# Autodesk Inventor assembly: Steam Engine Assembly
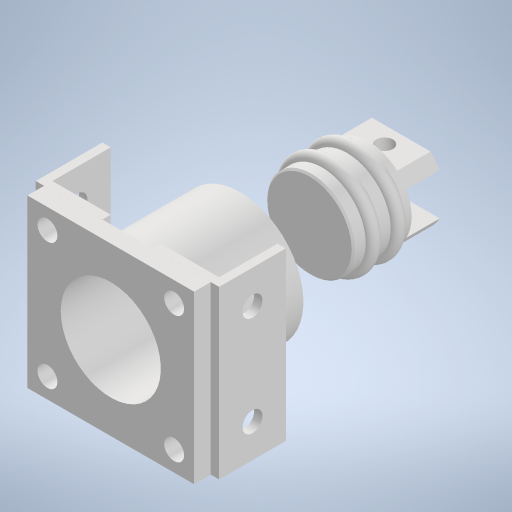
[picture p0: Inventor's stored thumbnail of the model, 512x512]
Saved by Autodesk Inventor 2023 (Build 270158000, 158)
## iProperties
Created: 2022-10-27
Part Number: Steam Engine Assembly
Document SubType Name: Assembly
Designer: tommy
Author: tommy
## Documents named in this file (5)
- C:\Users\tommy\Documents\Repositories\Steam Engine\Steam Engine Assembly.iam
- C:\Users\tommy\Documents\Repositories\Steam Engine\Cylinders.ipt
- C:\Users\tommy\Documents\Repositories\Steam Engine\Frame Bracket.ipt
- C:\Users\tommy\Documents\Repositories\Steam Engine\Piston.ipt
- C:\Users\tommy\Documents\Repositories\Steam Engine\Piston O Ring.ipt
## Components (6 placed, 4 different names)
1. Cylinders:1 — Mate:1, Mate:2, Mate:3, Mate:4, Mate:5, Mate:6, Mate:9
2. Frame Bracket:1 — Mate:1, Mate:3, Mate:4
3. Frame Bracket:2 — Mate:2, Mate:5, Mate:6
4. Piston:1 — Tangent:1, Tangent:2, Mate:7, Mate:8, Mate:9
5. Piston O Ring:1 — Tangent:2, Mate:8
6. Piston O Ring:2 — Tangent:1, Mate:7
## Relationships (11: Mate 9, Tangent 2)
- Mate:1: Cylinders:1 ↔ Frame Bracket:1
- Mate:2: Cylinders:1 ↔ Frame Bracket:2
- Mate:3: Cylinders:1 ↔ Frame Bracket:1
- Mate:4: Cylinders:1 ↔ Frame Bracket:1
- Mate:5: Cylinders:1 ↔ Frame Bracket:2
- Mate:6: Cylinders:1 ↔ Frame Bracket:2
- Tangent:1: Piston:1 ↔ Piston O Ring:2
- Tangent:2: Piston:1 ↔ Piston O Ring:1
- Mate:7: Piston:1 ↔ Piston O Ring:2
- Mate:8: Piston:1 ↔ Piston O Ring:1
- Mate:9: Cylinders:1 ↔ Piston:1
